# Autodesk Inventor assembly: HK0709FM
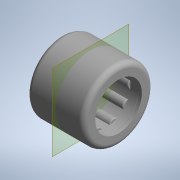
[picture p0: Inventor's stored thumbnail of the model, 180x180]
Saved by Autodesk Inventor 2020 (Build 240168000, 168)
## iProperties
Part Number: HK0709FM
Catalog Web Link: www.cadenas.de
Description: HK,HK..ZWD,HMK,HMK..ZWD (Open-end)-
Vendor: NTN
Document SubType Name: Assembly
Designer: partserver
Manufacturer: NTN
Mass: 0.362929 g
Surface Area: 14.1219 cm^2
Volume: 0.362929 cm^3
Density: 1 g/cm^3
Category: PARTsolutions
Company: NTN
PSOL_IDENT_0: {$CADENAS_DATA\23d-libs\ntn\needle_roler_bearings\needle_roller_shell_bearings\needle_roller_shell_b
PSOL_IDENT_1: earings_open_ended_asmtab.prj},198 {VTYP=3D},{STYP=ASSTAB},{NB=HK0709FM},{LINA=HK0709FM},{NN=HK,HK..
PSOL_IDENT_2: ZWD,HMK,HMK..ZWD (Open-end)},{DATE=29.01.2019 23:02:00},{GEOMDATE=13.08.2014 01:07:01},{VERSION=},{L
PSOL_IDENT_3: INEID=50},{WBVAR=},{WBNUMERIC=}  {NB=HK0709FM},{LINA=HK0709FM},{KT=DUMMY},{ORDER=HK0709FM},{FW=7},{D=
PSOL_IDENT_4: 11.0},{C=9},{CR=3150},{COR=2930},{CRF=320},{CORF=299},{LSG=23000},{LSO=34000},{MASS=0.0025},{IT=-},{
PSOL_IDENT_5: RT=1.6},{VER=1},{T=0.500},{DW=1.500},{LW=5.000},{NR=10.000},{CID=7.750},{CD=9.250},{CW=7.600},{SD=7.
PSOL_IDENT_6: 350},{PPATH=../needle_roller_shell_bearings_open_ended_asmtpl.prj}
NB: HK0709FM
NN: HK,HK..ZWD,HMK,HMK..ZWD (Open-end)
NBSYN: $ORDER.
LINA: HK0709FM
CATALOG: NTN Corporation
ORDER: HK0709FM
FW: 7
D: 11
C: 9
CR: 3150
COR: 2930
CRF: 320
CORF: 299
LSG: 23000
LSO: 34000
MASS: 0.0025
IT: -
SUPPLIER: NTN
ARTICLENO: HK0709FM
BOMINFO: HK0709FM
CREATOR: CADENAS GmbH
Title: HK0709FM
Author: Cadenas PARTsolutions
## Documents named in this file (4)
- C:\Users\avi41\Desktop\Robot Arm\CAD_files\HK0709FM.iam
- C:\Users\avi41\Desktop\Robot Arm\CAD_files\HK0709FMSH.ipt
- C:\Users\avi41\Desktop\Robot Arm\CAD_files\HK0709FMCA.ipt
- C:\Users\avi41\Desktop\Robot Arm\CAD_files\HK0709FMRO.ipt
## Components (12 placed, 3 different names)
1. HK0709FMSH:1 — IP_5_XY@1 <-> IP_1_XY@2, IP_5_Z@1 <-> IP_1_Z@2, Symmetry:1
2. HK0709FMCA:1 — IP_5_XY@1 <-> IP_1_XY@2, IP_5_Z@1 <-> IP_1_Z@2, IP_3_1_XY@2 <-> IP_1_XY@3, IP_3_1_Z@2 <-> IP_1_Z@3, IP_3_1_YZ@2 <-> IP_1_YZ@3, IP_3_2_XY@2 <-> IP_1_XY@4, IP_3_2_Z@2 <-> IP_1_Z@4, IP_3_2_YZ@2 <-> IP_1_YZ@4, IP_3_3_XY@2 <-> IP_1_XY@5, IP_3_3_Z@2 <-> IP_1_Z@5, IP_3_3_YZ@2 <-> IP_1_YZ@5, IP_3_4_XY@2 <-> IP_1_XY@6, IP_3_4_Z@2 <-> IP_1_Z@6, IP_3_4_YZ@2 <-> IP_1_YZ@6, IP_3_5_XY@2 <-> IP_1_XY@7, IP_3_5_Z@2 <-> IP_1_Z@7, IP_3_5_YZ@2 <-> IP_1_YZ@7, IP_3_6_XY@2 <-> IP_1_XY@8, IP_3_6_Z@2 <-> IP_1_Z@8, IP_3_6_YZ@2 <-> IP_1_YZ@8, IP_3_7_XY@2 <-> IP_1_XY@9, IP_3_7_Z@2 <-> IP_1_Z@9, IP_3_7_YZ@2 <-> IP_1_YZ@9, IP_3_8_XY@2 <-> IP_1_XY@10, IP_3_8_Z@2 <-> IP_1_Z@10, IP_3_8_YZ@2 <-> IP_1_YZ@10, IP_3_9_XY@2 <-> IP_1_XY@11, IP_3_9_Z@2 <-> IP_1_Z@11, IP_3_9_YZ@2 <-> IP_1_YZ@11, IP_3_10_XY@2 <-> IP_1_XY@12, IP_3_10_Z@2 <-> IP_1_Z@12, IP_3_10_YZ@2 <-> IP_1_YZ@12, Symmetry:1
3. HK0709FMRO:1 — IP_3_1_XY@2 <-> IP_1_XY@3, IP_3_1_Z@2 <-> IP_1_Z@3, IP_3_1_YZ@2 <-> IP_1_YZ@3
4. HK0709FMRO:2 — IP_3_2_XY@2 <-> IP_1_XY@4, IP_3_2_Z@2 <-> IP_1_Z@4, IP_3_2_YZ@2 <-> IP_1_YZ@4
5. HK0709FMRO:3 — IP_3_3_XY@2 <-> IP_1_XY@5, IP_3_3_Z@2 <-> IP_1_Z@5, IP_3_3_YZ@2 <-> IP_1_YZ@5
6. HK0709FMRO:4 — IP_3_4_XY@2 <-> IP_1_XY@6, IP_3_4_Z@2 <-> IP_1_Z@6, IP_3_4_YZ@2 <-> IP_1_YZ@6
7. HK0709FMRO:5 — IP_3_5_XY@2 <-> IP_1_XY@7, IP_3_5_Z@2 <-> IP_1_Z@7, IP_3_5_YZ@2 <-> IP_1_YZ@7
8. HK0709FMRO:6 — IP_3_6_XY@2 <-> IP_1_XY@8, IP_3_6_Z@2 <-> IP_1_Z@8, IP_3_6_YZ@2 <-> IP_1_YZ@8
9. HK0709FMRO:7 — IP_3_7_XY@2 <-> IP_1_XY@9, IP_3_7_Z@2 <-> IP_1_Z@9, IP_3_7_YZ@2 <-> IP_1_YZ@9
10. HK0709FMRO:8 — IP_3_8_XY@2 <-> IP_1_XY@10, IP_3_8_Z@2 <-> IP_1_Z@10, IP_3_8_YZ@2 <-> IP_1_YZ@10
11. HK0709FMRO:9 — IP_3_9_XY@2 <-> IP_1_XY@11, IP_3_9_Z@2 <-> IP_1_Z@11, IP_3_9_YZ@2 <-> IP_1_YZ@11
12. HK0709FMRO:10 — IP_3_10_XY@2 <-> IP_1_XY@12, IP_3_10_Z@2 <-> IP_1_Z@12, IP_3_10_YZ@2 <-> IP_1_YZ@12
## Relationships (33: Mate 21, Angle 10, Flush 1, Symmetry 1)
- IP_5_XY@1 <-> IP_1_XY@2 [Flush]: HK0709FMSH:1 ↔ HK0709FMCA:1
- IP_5_Z@1 <-> IP_1_Z@2 [Mate]: HK0709FMSH:1 ↔ HK0709FMCA:1
- IP_3_1_XY@2 <-> IP_1_XY@3 [Mate]: HK0709FMCA:1 ↔ HK0709FMRO:1
- IP_3_1_Z@2 <-> IP_1_Z@3 [Mate]: HK0709FMCA:1 ↔ HK0709FMRO:1
- IP_3_1_YZ@2 <-> IP_1_YZ@3 [Angle] (0 deg): HK0709FMCA:1 ↔ HK0709FMRO:1
- IP_3_2_XY@2 <-> IP_1_XY@4 [Mate]: HK0709FMCA:1 ↔ HK0709FMRO:2
- IP_3_2_Z@2 <-> IP_1_Z@4 [Mate]: HK0709FMCA:1 ↔ HK0709FMRO:2
- IP_3_2_YZ@2 <-> IP_1_YZ@4 [Angle] (0 deg): HK0709FMCA:1 ↔ HK0709FMRO:2
- IP_3_3_XY@2 <-> IP_1_XY@5 [Mate]: HK0709FMCA:1 ↔ HK0709FMRO:3
- IP_3_3_Z@2 <-> IP_1_Z@5 [Mate]: HK0709FMCA:1 ↔ HK0709FMRO:3
- IP_3_3_YZ@2 <-> IP_1_YZ@5 [Angle] (0 deg): HK0709FMCA:1 ↔ HK0709FMRO:3
- IP_3_4_XY@2 <-> IP_1_XY@6 [Mate]: HK0709FMCA:1 ↔ HK0709FMRO:4
- IP_3_4_Z@2 <-> IP_1_Z@6 [Mate]: HK0709FMCA:1 ↔ HK0709FMRO:4
- IP_3_4_YZ@2 <-> IP_1_YZ@6 [Angle] (0 deg): HK0709FMCA:1 ↔ HK0709FMRO:4
- IP_3_5_XY@2 <-> IP_1_XY@7 [Mate]: HK0709FMCA:1 ↔ HK0709FMRO:5
- IP_3_5_Z@2 <-> IP_1_Z@7 [Mate]: HK0709FMCA:1 ↔ HK0709FMRO:5
- IP_3_5_YZ@2 <-> IP_1_YZ@7 [Angle] (0 deg): HK0709FMCA:1 ↔ HK0709FMRO:5
- IP_3_6_XY@2 <-> IP_1_XY@8 [Mate]: HK0709FMCA:1 ↔ HK0709FMRO:6
- IP_3_6_Z@2 <-> IP_1_Z@8 [Mate]: HK0709FMCA:1 ↔ HK0709FMRO:6
- IP_3_6_YZ@2 <-> IP_1_YZ@8 [Angle] (0 deg): HK0709FMCA:1 ↔ HK0709FMRO:6
- IP_3_7_XY@2 <-> IP_1_XY@9 [Mate]: HK0709FMCA:1 ↔ HK0709FMRO:7
- IP_3_7_Z@2 <-> IP_1_Z@9 [Mate]: HK0709FMCA:1 ↔ HK0709FMRO:7
- IP_3_7_YZ@2 <-> IP_1_YZ@9 [Angle] (0 deg): HK0709FMCA:1 ↔ HK0709FMRO:7
- IP_3_8_XY@2 <-> IP_1_XY@10 [Mate]: HK0709FMCA:1 ↔ HK0709FMRO:8
- IP_3_8_Z@2 <-> IP_1_Z@10 [Mate]: HK0709FMCA:1 ↔ HK0709FMRO:8
- IP_3_8_YZ@2 <-> IP_1_YZ@10 [Angle] (0 deg): HK0709FMCA:1 ↔ HK0709FMRO:8
- IP_3_9_XY@2 <-> IP_1_XY@11 [Mate]: HK0709FMCA:1 ↔ HK0709FMRO:9
- IP_3_9_Z@2 <-> IP_1_Z@11 [Mate]: HK0709FMCA:1 ↔ HK0709FMRO:9
- IP_3_9_YZ@2 <-> IP_1_YZ@11 [Angle] (0 deg): HK0709FMCA:1 ↔ HK0709FMRO:9
- IP_3_10_XY@2 <-> IP_1_XY@12 [Mate]: HK0709FMCA:1 ↔ HK0709FMRO:10
- IP_3_10_Z@2 <-> IP_1_Z@12 [Mate]: HK0709FMCA:1 ↔ HK0709FMRO:10
- IP_3_10_YZ@2 <-> IP_1_YZ@12 [Angle] (0 deg): HK0709FMCA:1 ↔ HK0709FMRO:10
- Symmetry:1: HK0709FMSH:1 ↔ HK0709FMCA:1
